# Autodesk Inventor assembly: 206.001.01_Schieberbetaetigung
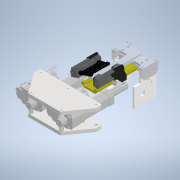
[picture p0: Inventor's stored thumbnail of the model, 180x180]
Saved by Autodesk Inventor 2022 (Build 260153000, 153)
## iProperties
Created: 2021-11-14
Part Number: 206.001.01_Schieberbetaetigung
Document SubType Name: Assembly
Designer: Oliver Ungerer
KODE_ZEICHNUNGSNUMMER: TFVEM_110M
BENENNUNG: Fuehrung Schieber
BEARBEITER_NAME: Ungerer O.
MASSE: 2.190774
PDMREV: 0.0+
PDMRL: Entwicklung
PROI_REVISION: 0
PROI_VERSION: 0+
PROI_RELEASE: Entwicklung
PTC_MODIFIED: True
PROI_CREATED_BY: Kantioler_adm
PROI_CREATED_ON: 07.03.2008 12:11:19
PROI_LOCATION: Root-Ordner/Pro_stds/Start_Files
MATERIALART: -
EINHEIT: ST
HERSTELLER_PREIS: 0.0
PRUEFER_NAME: Uo
PTC_ORGANIZATION_ID: Durst
PTC_WM_REVISION: 0
PTC_WM_ITERATION: 0
PTC_WM_VERSION: 0.0
PTC_WM_LIFECYCLE_STATE: Entwicklung
PTC_WM_LIFECYCLE: 02 Durst
PTC_WM_CREATED_BY: Oliver Ungerer (oungerer: Durst)
PTC_WM_CREATED_ON: 01.08.21
PTC_WM_MODIFIED_BY: Oliver Ungerer (oungerer: Durst)
PTC_WM_MODIFIED_ON: 01.08.21
AEND_INDEX: 0
VERSION: 0
STATUS: 0.0
Author: Oliver Ungerer
## Documents named in this file (17)
- C:\Users\kaebi\OneDrive - mci4me.at\03_MCI Master\4.Semester_SS2022\Masterarbeit\Software\CAD\106_Vereinzelungseinheit\206.002.01_Schieberbetaetigung.iam
- C:\Users\kaebi\OneDrive - mci4me.at\03_MCI Master\4.Semester_SS2022\Masterarbeit\Software\CAD\106_Vereinzelungseinheit\506.004.01_IGUS_Schiene.ipt
- C:\Users\kaebi\OneDrive - mci4me.at\03_MCI Master\4.Semester_SS2022\Masterarbeit\Software\CAD\106_Vereinzelungseinheit\106.016.01_Schienenfuehrung.ipt
- C:\Users\kaebi\OneDrive - mci4me.at\03_MCI Master\4.Semester_SS2022\Masterarbeit\Software\CAD\106_Vereinzelungseinheit\106.019.01_Distanzplatte.ipt
- C:\Users\kaebi\OneDrive - mci4me.at\03_MCI Master\4.Semester_SS2022\Masterarbeit\Software\CAD\106_Vereinzelungseinheit\106.018.01_Schieberelement_oben.ipt
- C:\Users\kaebi\OneDrive - mci4me.at\03_MCI Master\4.Semester_SS2022\Masterarbeit\Software\CAD\106_Vereinzelungseinheit\106.020.01_Winkelaufnahme_Schwert_unten.ipt
- C:\Users\kaebi\OneDrive - mci4me.at\03_MCI Master\4.Semester_SS2022\Masterarbeit\Software\CAD\106_Vereinzelungseinheit\106.030.01_Schwert_oben.ipt
- C:\Users\kaebi\OneDrive - mci4me.at\03_MCI Master\4.Semester_SS2022\Masterarbeit\Software\CAD\106_Vereinzelungseinheit\106.033.01_Schwert_unten.ipt
- C:\Users\kaebi\OneDrive - mci4me.at\03_MCI Master\4.Semester_SS2022\Masterarbeit\Software\CAD\106_Vereinzelungseinheit\206.003.02_Kraftlimitierung.iam
- C:\Users\kaebi\OneDrive - mci4me.at\03_MCI Master\4.Semester_SS2022\Masterarbeit\Software\CAD\106_Vereinzelungseinheit\206.004.02_Kraftlimitierung.iam
- C:\Users\kaebi\OneDrive - mci4me.at\03_MCI Master\4.Semester_SS2022\Masterarbeit\Software\CAD\106_Vereinzelungseinheit\506.007.01_Linearaktor.iam
- C:\Users\kaebi\OneDrive - mci4me.at\03_MCI Master\4.Semester_SS2022\Masterarbeit\Software\CAD\106_Vereinzelungseinheit\106.023.01_Zapfen_Aktor.ipt
- C:\Users\kaebi\OneDrive - mci4me.at\03_MCI Master\4.Semester_SS2022\Masterarbeit\Software\CAD\106_Vereinzelungseinheit\106.024.01_Zapfen_Aktor_Auflage.ipt
- C:\Users\kaebi\OneDrive - mci4me.at\03_MCI Master\4.Semester_SS2022\Masterarbeit\Software\CAD\106_Vereinzelungseinheit\106.025.01_Anbindung_Aktor.ipt
- C:\Users\kaebi\OneDrive - mci4me.at\03_MCI Master\4.Semester_SS2022\Masterarbeit\Software\CAD\106_Vereinzelungseinheit\106.034.01_Schieberelement_unten.ipt
- C:\Users\kaebi\OneDrive - mci4me.at\03_MCI Master\4.Semester_SS2022\Masterarbeit\Software\CAD\106_Vereinzelungseinheit\SchlittenUnten.iam
- C:\Users\kaebi\OneDrive - mci4me.at\03_MCI Master\4.Semester_SS2022\Masterarbeit\Software\CAD\106_Vereinzelungseinheit\SchlittenOben.iam
## Components (25 placed, 16 different names)
1. 506.004.01_IGUS_Schiene — Fluchtend:1, Passend:15, Winkel:1, Passend:20, Winkel:2, Fluchtend:2, Passend:21, Winkel:3, Passend:23, Winkel:4, Fluchtend:69, Winkel:5, Passend:86, Passend:87, Passend:89, Passend:90
2. 506.007.01_Linearaktor [sub-assembly] — Passend:1, Passend:2, Fluchtend:70, Passend:88
3. 506.007.01_Linearaktor:2 [sub-assembly] — Fluchtend:69, Winkel:5, Passend:68, Passend:69, Fluchtend:70, Passend:91
4. 106.023.01_Zapfen_Aktor — Passend:7, Passend:8, Passend:68, Passend:69, Passend:71
5. 106.023.01_Zapfen_Aktor:1 — Passend:1, Passend:2, Passend:5, Passend:6, Passend:72, Passend:73
6. 106.024.01_Zapfen_Aktor_Auflage — Passend:7, Passend:8
7. 106.024.01_Zapfen_Aktor_Auflage:1 — Passend:5, Passend:6
8. 106.025.01_Anbindung_Aktor — Passend:71, Passend:72, Passend:73, Winkel:6
9. 106.025.01_Anbindung_Aktor:1
10. SchlittenUnten:1 [sub-assembly] — Passend:86, Passend:87, Passend:88
11. SchlittenOben:1 [sub-assembly] — Passend:89, Passend:90, Passend:91
12. 106.016.01_Schienenfuehrung:1 — Passend:22, Passend:23, Winkel:4, Passend:26, Passend:75, Passend:76, Passend:80
13. 106.019.01_Distanzplatte:1 — Passend:26, Passend:75, Passend:76
14. 106.016.01_Schienenfuehrung — Fluchtend:1, Passend:15, Winkel:1, Passend:18, Passend:19, Passend:77, Passend:78
15. 106.019.01_Distanzplatte — Passend:18, Passend:29, Passend:77, Passend:78, Passend:79
16. 106.018.01_Schieberelement_oben — Passend:29, Passend:36, Passend:37, Passend:38, Passend:50, Passend:79, Passend:80, Winkel:6, Passend:83, Passend:84
17. 106.020.01_Winkelaufnahme_Schwert_unten — Passend:36, Passend:37, Passend:38, Passend:44, Passend:85, Fluchtend:71
18. 106.030.01_Schwert_oben — Passend:44, Passend:85, Fluchtend:71
19. 206.004.02_Kraftlimitierung [sub-assembly] — Passend:50, Passend:83, Passend:84
20. 206.003.02_Kraftlimitierung [sub-assembly] — Passend:47, Passend:81, Passend:82
21. 106.016.01_Schienenfuehrung:2 — Fluchtend:2, Passend:21, Winkel:3, Passend:22, Passend:32, Passend:74
22. 106.016.01_Schienenfuehrung:3 — Passend:19, Passend:20, Winkel:2, Passend:31
23. 106.034.01_Schieberelement_unten:1 — Passend:31, Passend:32, Passend:33, Passend:34, Passend:35, Passend:47, Passend:74, Passend:81, Passend:82
24. 106.020.01_Winkelaufnahme_Schwert_unten:1 — Passend:33, Passend:34, Passend:35, Passend:39, Passend:40, Passend:41
25. 106.033.01_Schwert_unten — Passend:39, Passend:40, Passend:41
## Relationships (66: Mate 55, Angle 6, Flush 5)
- Passend:1 [Mate] (1 mm): 506.007.01_Linearaktor ↔ 106.023.01_Zapfen_Aktor:1
- Passend:2 [Mate]: 506.007.01_Linearaktor ↔ 106.023.01_Zapfen_Aktor:1
- Passend:5 [Mate]: 106.023.01_Zapfen_Aktor:1 ↔ 106.024.01_Zapfen_Aktor_Auflage:1
- Passend:6 [Mate]: 106.023.01_Zapfen_Aktor:1 ↔ 106.024.01_Zapfen_Aktor_Auflage:1
- Passend:7 [Mate]: 106.023.01_Zapfen_Aktor ↔ 106.024.01_Zapfen_Aktor_Auflage
- Passend:8 [Mate]: 106.023.01_Zapfen_Aktor ↔ 106.024.01_Zapfen_Aktor_Auflage
- [Mate]: 106.024.01_Zapfen_Aktor_Auflage:1 ↔ 106.025.01_Anbindung_Aktor:1
- [Mate]: 106.024.01_Zapfen_Aktor_Auflage ↔ 106.025.01_Anbindung_Aktor:1
- [Mate]: 106.024.01_Zapfen_Aktor_Auflage:1 ↔ 106.025.01_Anbindung_Aktor:1
- Fluchtend:1 [Flush] (0.5 mm): 506.004.01_IGUS_Schiene ↔ 106.016.01_Schienenfuehrung
- Passend:15 [Mate]: 506.004.01_IGUS_Schiene ↔ 106.016.01_Schienenfuehrung
- Winkel:1 [Angle] (0 deg): 506.004.01_IGUS_Schiene ↔ 106.016.01_Schienenfuehrung
- Passend:18 [Mate]: 106.016.01_Schienenfuehrung ↔ 106.019.01_Distanzplatte
- Passend:19 [Mate] (51 mm): 106.016.01_Schienenfuehrung ↔ 106.016.01_Schienenfuehrung:3
- Passend:20 [Mate]: 506.004.01_IGUS_Schiene ↔ 106.016.01_Schienenfuehrung:3
- Winkel:2 [Angle] (0 deg): 506.004.01_IGUS_Schiene ↔ 106.016.01_Schienenfuehrung:3
- Fluchtend:2 [Flush] (0.5 mm): 506.004.01_IGUS_Schiene ↔ 106.016.01_Schienenfuehrung:2
- Passend:21 [Mate]: 506.004.01_IGUS_Schiene ↔ 106.016.01_Schienenfuehrung:2
- Winkel:3 [Angle] (0 deg): 506.004.01_IGUS_Schiene ↔ 106.016.01_Schienenfuehrung:2
- Passend:22 [Mate] (51 mm): 106.016.01_Schienenfuehrung:1 ↔ 106.016.01_Schienenfuehrung:2
- Passend:23 [Mate]: 506.004.01_IGUS_Schiene ↔ 106.016.01_Schienenfuehrung:1
- Winkel:4 [Angle] (0 deg): 506.004.01_IGUS_Schiene ↔ 106.016.01_Schienenfuehrung:1
- Passend:26 [Mate]: 106.016.01_Schienenfuehrung:1 ↔ 106.019.01_Distanzplatte:1
- Passend:29 [Mate]: 106.019.01_Distanzplatte ↔ 106.018.01_Schieberelement_oben
- Passend:31 [Mate]: 106.016.01_Schienenfuehrung:3 ↔ 106.034.01_Schieberelement_unten:1
- Passend:32 [Mate]: 106.016.01_Schienenfuehrung:2 ↔ 106.034.01_Schieberelement_unten:1
- Passend:33 [Mate]: 106.034.01_Schieberelement_unten:1 ↔ 106.020.01_Winkelaufnahme_Schwert_unten:1
- Passend:34 [Mate]: 106.034.01_Schieberelement_unten:1 ↔ 106.020.01_Winkelaufnahme_Schwert_unten:1
- Passend:35 [Mate]: 106.034.01_Schieberelement_unten:1 ↔ 106.020.01_Winkelaufnahme_Schwert_unten:1
- Passend:36 [Mate]: 106.018.01_Schieberelement_oben ↔ 106.020.01_Winkelaufnahme_Schwert_unten
- Passend:37 [Mate]: 106.018.01_Schieberelement_oben ↔ 106.020.01_Winkelaufnahme_Schwert_unten
- Passend:38 [Mate]: 106.018.01_Schieberelement_oben ↔ 106.020.01_Winkelaufnahme_Schwert_unten
- Passend:39 [Mate]: 106.020.01_Winkelaufnahme_Schwert_unten:1 ↔ 106.033.01_Schwert_unten
- Passend:40 [Mate]: 106.020.01_Winkelaufnahme_Schwert_unten:1 ↔ 106.033.01_Schwert_unten
- Passend:41 [Mate]: 106.020.01_Winkelaufnahme_Schwert_unten:1 ↔ 106.033.01_Schwert_unten
- Passend:44 [Mate]: 106.020.01_Winkelaufnahme_Schwert_unten ↔ 106.030.01_Schwert_oben
- Passend:47 [Mate]: 206.003.02_Kraftlimitierung ↔ 106.034.01_Schieberelement_unten:1
- Passend:50 [Mate]: 106.018.01_Schieberelement_oben ↔ 206.004.02_Kraftlimitierung
- Fluchtend:69 [Flush] (6 mm): 506.004.01_IGUS_Schiene ↔ 506.007.01_Linearaktor:2
- Winkel:5 [Angle] (0 deg): 506.004.01_IGUS_Schiene ↔ 506.007.01_Linearaktor:2
- Passend:68 [Mate]: 506.007.01_Linearaktor:2 ↔ 106.023.01_Zapfen_Aktor
- Passend:69 [Mate] (1 mm): 506.007.01_Linearaktor:2 ↔ 106.023.01_Zapfen_Aktor
- Fluchtend:70 [Flush]: 506.007.01_Linearaktor ↔ 506.007.01_Linearaktor:2
- Passend:71 [Mate]: 106.023.01_Zapfen_Aktor ↔ 106.025.01_Anbindung_Aktor
- Passend:72 [Mate]: 106.023.01_Zapfen_Aktor:1 ↔ 106.025.01_Anbindung_Aktor
- Passend:73 [Mate]: 106.023.01_Zapfen_Aktor:1 ↔ 106.025.01_Anbindung_Aktor
- Passend:74 [Mate]: 106.016.01_Schienenfuehrung:2 ↔ 106.034.01_Schieberelement_unten:1
- Passend:75 [Mate]: 106.016.01_Schienenfuehrung:1 ↔ 106.019.01_Distanzplatte:1
- Passend:76 [Mate]: 106.016.01_Schienenfuehrung:1 ↔ 106.019.01_Distanzplatte:1
- Passend:77 [Mate]: 106.016.01_Schienenfuehrung ↔ 106.019.01_Distanzplatte
- Passend:78 [Mate]: 106.016.01_Schienenfuehrung ↔ 106.019.01_Distanzplatte
- Passend:79 [Mate]: 106.019.01_Distanzplatte ↔ 106.018.01_Schieberelement_oben
- Passend:80 [Mate]: 106.016.01_Schienenfuehrung:1 ↔ 106.018.01_Schieberelement_oben
- Winkel:6 [Angle] (0 deg): 106.025.01_Anbindung_Aktor ↔ 106.018.01_Schieberelement_oben
- Passend:81 [Mate]: 206.003.02_Kraftlimitierung ↔ 106.034.01_Schieberelement_unten:1
- Passend:82 [Mate]: 206.003.02_Kraftlimitierung ↔ 106.034.01_Schieberelement_unten:1
- Passend:83 [Mate]: 106.018.01_Schieberelement_oben ↔ 206.004.02_Kraftlimitierung
- Passend:84 [Mate]: 106.018.01_Schieberelement_oben ↔ 206.004.02_Kraftlimitierung
- Passend:85 [Mate]: 106.020.01_Winkelaufnahme_Schwert_unten ↔ 106.030.01_Schwert_oben
- Fluchtend:71 [Flush]: 106.020.01_Winkelaufnahme_Schwert_unten ↔ 106.030.01_Schwert_oben
- Passend:86 [Mate]: 506.004.01_IGUS_Schiene ↔ SchlittenUnten:1
- Passend:87 [Mate]: 506.004.01_IGUS_Schiene ↔ SchlittenUnten:1
- Passend:88 [Mate]: 506.007.01_Linearaktor ↔ SchlittenUnten:1
- Passend:89 [Mate]: 506.004.01_IGUS_Schiene ↔ SchlittenOben:1
- Passend:90 [Mate]: 506.004.01_IGUS_Schiene ↔ SchlittenOben:1
- Passend:91 [Mate]: 506.007.01_Linearaktor:2 ↔ SchlittenOben:1
## Named parameters: d11_d6 = 0 mm, d12_d7 = 0 mm
